# Autodesk Inventor assembly: Front_Train
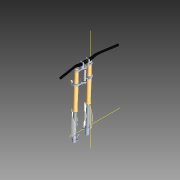
[picture p0: Inventor's stored thumbnail of the model, 180x180]
Saved by Autodesk Inventor 2016 (Build 200138000, 138)
## iProperties
Created: 2015-04-04
Part Number: Front_Train
Document SubType Name: Assembly
Designer: Yann
Author: Yann
## iProperties of the stored document Handlebar.ipt
Created: 2014-11-08
Part Number: Handlebar
Material: Generic
Document SubType Name: Modeling
Designer: Yann
Density: 1 g/cm^3
Appearance: Default
Sending System: SolidWorks 2012
Last Author: Stormtrooper
Last Saved: 2014-11-19
Author: Yann
## Documents named in this file (4)
- **C:\Users\Yann\Documents\GitHub\BIKAIR_CAD\Source\Front_Train\Front_Train.iam*LocalDocs*xOqdabbqfCq0wujc0Oz4mrtfs3b*Handlebar.ipt
- C:\Users\Yann\Documents\GitHub\BIKAIR_CAD\Source\Front_Train\Front_Train.iam
- C:\Users\Yann\Documents\GitHub\BIKAIR_CAD\Source\Front_Train\Fork\Scaled_CR85_Fork.ipt
- C:\Users\Yann\Documents\GitHub\BIKAIR_CAD\Source\Front_Train\Handlebar.SLDPRT
## Components (2 placed, 2 different names)
1. Scaled_CR85_Fork:1 — Mate:10, Mate:11, Mate:12
2. Handlebar:2 — Mate:12, Mate:13
## Relationships (5: Mate 5)
- Mate:7
- Mate:10: Scaled_CR85_Fork:1
- Mate:11: Scaled_CR85_Fork:1
- Mate:12: Scaled_CR85_Fork:1 ↔ Handlebar:2
- Mate:13: Handlebar:2
